# Autodesk Inventor assembly: Assembly2
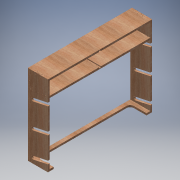
[picture p0: Inventor's stored thumbnail of the model, 180x180]
Saved by Autodesk Inventor 2016 (Build 200138000, 138)
## iProperties
Created: 2017-03-13
Part Number: Assembly2
Document SubType Name: Assembly
Designer: jwillauer
Author: jwillauer
## Documents named in this file (6)
- C:\Users\jwillauer\Desktop\make something big folder\Assembly2.iam
- C:\Users\jwillauer\Desktop\make something big folder\rack sides.ipt
- C:\Users\jwillauer\Desktop\make something big folder\top.ipt
- C:\Users\jwillauer\Desktop\make something big folder\shelf.ipt
- C:\Users\jwillauer\Desktop\make something big folder\bottom.ipt
- C:\Users\jwillauer\Desktop\make something big folder\shelf back.ipt
## Components (6 placed, 5 different names)
1. rack sides:1 — Flush:3, Flush:4, Mate:2, Flush:5, Mate:3, Flush:6, Mate:4, Flush:7, Mate:5, Mate:6, Mate:8
2. rack sides:2 — Mate:1, Flush:1, Flush:2, Mate:7, Flush:8
3. top:1 — Mate:1, Flush:1, Flush:2, Flush:3, Flush:4, Mate:6
4. shelf:1 — Mate:2, Flush:5, Mate:3, Flush:6, Mate:9
5. bottom:1 — Mate:4, Flush:7, Mate:5
6. shelf back:1 — Mate:7, Flush:8, Mate:8, Mate:9
## Relationships (17: Mate 9, Flush 8)
- Mate:1: rack sides:2 ↔ top:1
- Flush:1: rack sides:2 ↔ top:1
- Flush:2: rack sides:2 ↔ top:1
- Flush:3: rack sides:1 ↔ top:1
- Flush:4: rack sides:1 ↔ top:1
- Mate:2: rack sides:1 ↔ shelf:1
- Flush:5: rack sides:1 ↔ shelf:1
- Mate:3: rack sides:1 ↔ shelf:1
- Flush:6: rack sides:1 ↔ shelf:1
- Mate:4: rack sides:1 ↔ bottom:1
- Flush:7: rack sides:1 ↔ bottom:1
- Mate:5: rack sides:1 ↔ bottom:1
- Mate:6: rack sides:1 ↔ top:1
- Mate:7: rack sides:2 ↔ shelf back:1
- Flush:8: rack sides:2 ↔ shelf back:1
- Mate:8: rack sides:1 ↔ shelf back:1
- Mate:9: shelf:1 ↔ shelf back:1
